# Autodesk Inventor assembly: Estructura_02
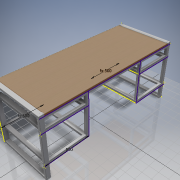
[picture p0: Inventor's stored thumbnail of the model, 180x180]
Saved by Autodesk Inventor 2016 (Build 200138000, 138)
## iProperties
Created: 2018-06-24
Part Number: Estructura_02
Document SubType Name: Assembly
Designer: damia
_SolveAssemblyDoc: Frame Generator Solve Assembly
_Version: 15.0.0
Author: damia
## Documents named in this file (5)
- C:\Users\damia\Documents\Inventor\escritorio_Damian\Estructura_02.iam
- C:\Users\damia\Documents\Inventor\escritorio_Damian\Esqueleto.ipt
- C:\Users\damia\Documents\Inventor\escritorio_Damian\Estructura\Frame\Frame0001.iam
- C:\Users\damia\Documents\Inventor\escritorio_Damian\tapa.ipt
- C:\Users\damia\Documents\Inventor\escritorio_Damian\vidro.ipt
## Components (4 placed, 4 different names)
1. Esqueleto:1
2. Frame0001:1 [sub-assembly] — Flush:1, Mate:1, Mate:2, Mate:3
3. tapa:1 — Flush:1, Mate:1, Mate:2, Flush:2, Mate:4
4. vidro:1 — Mate:3, Flush:2, Mate:4
## Relationships (6: Mate 4, Flush 2)
- Flush:1: Frame0001:1 ↔ tapa:1
- Mate:1: Frame0001:1 ↔ tapa:1
- Mate:2: Frame0001:1 ↔ tapa:1
- Mate:3: Frame0001:1 ↔ vidro:1
- Flush:2: tapa:1 ↔ vidro:1
- Mate:4: tapa:1 ↔ vidro:1
